# Autodesk Inventor assembly: High Strength 60-Tooth Gear-With High Strength Square Gear Insert
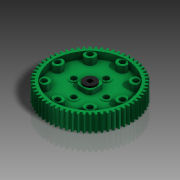
[picture p0: Inventor's stored thumbnail of the model, 180x180]
Saved by Autodesk Inventor 2016 (Build 200138000, 138)
## iProperties
Created: 2010-10-31
Part Number: High Strength 60-Tooth Gear-With High Strength Square Gear Insert
Document SubType Name: Assembly
Designer: JordanK
Author: JordanK
## Documents named in this file (3)
- D:\New Laptop\(1) New Laptop\AFNAN ALI flashdrive backup\VEXPARTS\Vex parts\Gears & Pulleys\High Strength 60-Tooth Gear-With High Strength Square Gear Insert.iam
- D:\New Laptop\(1) New Laptop\AFNAN ALI flashdrive backup\VEXPARTS\Vex parts\Gears & Pulleys\High Strength 60-Tooth Gear.ipt
- D:\New Laptop\(1) New Laptop\AFNAN ALI flashdrive backup\VEXPARTS\Vex parts\Gears & Pulleys\High Strength Square Gear Insert.ipt
## Components (3 placed, 2 different names)
1. High Strength 60-Tooth Gear:1 — Mate:1, Mate:2, Mate:3, Mate:4
2. High Strength Square Gear Insert:1 — Mate:1, Mate:2
3. High Strength Square Gear Insert:2 — Mate:3, Mate:4
## Relationships (4: Mate 4)
- Mate:1: High Strength 60-Tooth Gear:1 ↔ High Strength Square Gear Insert:1
- Mate:2: High Strength 60-Tooth Gear:1 ↔ High Strength Square Gear Insert:1
- Mate:3: High Strength 60-Tooth Gear:1 ↔ High Strength Square Gear Insert:2
- Mate:4: High Strength 60-Tooth Gear:1 ↔ High Strength Square Gear Insert:2
